# Autodesk Inventor assembly: HOATrap
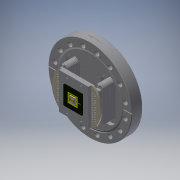
[picture p0: Inventor's stored thumbnail of the model, 180x180]
Saved by Autodesk Inventor 2016 (Build 200138000, 138)
## iProperties
Created: 2013-12-11
Part Number: HOATrap
Document SubType Name: Assembly
Designer: Michael
Author: Michael
## Documents named in this file (9)
- C:\Users\Michael\Dropbox (Personal)\Code\CAD---Experiment-systems\twins\Experiment flange\HOATrap.iam
- C:\Users\Michael\Dropbox\DO_NOT_DELETE\Flanges\Feedthroughs\Imported Components\6in_Custom_100pin\6in_Custom_100pin_Mounting_2.ipt
- C:\Users\Michael\Dropbox\DO_NOT_DELETE\UHV wiring\UHVPCB\SandiaWireRouting.ipt
- C:\Users\Michael\Dropbox\DO_NOT_DELETE\UHV wiring\mill-max-0461-3-15-15-21-XX-04-0.iam
- C:\Users\Michael\Dropbox\DO_NOT_DELETE\Flanges\Windows\Imported Components\133in_SapphireWindow_KL\133in_SapphireWindow_KL.iam
- C:\Users\Michael\Dropbox\DO_NOT_DELETE\UHV wiring\mill-max-3136-2-00-15-00-00-08-0.ipt
- C:\Users\Michael\Dropbox\DO_NOT_DELETE\Electronics\Connectors\dbConnectors\db50\db50UHV_adapter.iam
- C:\Users\Michael\Dropbox\DO_NOT_DELETE\Trap Designs\Sandia HOA Trap\HOA-Trap_Assembly.iam
- C:\Users\Michael\Dropbox (MIT)\Quanta\MG\CAD\Experiment\CavityMount.ipt
## Components (207 placed, 8 different names)
1. 6in_Custom_100pin_Mounting_2:1 — Insert:1, Angle:1, Insert:11, Insert:22, Insert:23, Insert:24, Insert:25
2. SandiaWireRouting:1 — Insert:1, Angle:1, Insert:2, Insert:12, Insert:13, Insert:14, Insert:15, Insert:16, Insert:17, Insert:18, Insert:19, Insert:20, Insert:21, Insert:28, Insert:29
3. HOA-Trap_Assembly:1 [sub-assembly] — Insert:3, Insert:4
4. 133in_SapphireWindow_KL:1 [sub-assembly] — Insert:11
5. mill-max-3136-2-00-15-00-00-08-0:50 — Insert:19
6. mill-max-3136-2-00-15-00-00-08-0:54 — Insert:18
7. mill-max-3136-2-00-15-00-00-08-0:100 — Insert:21
8. mill-max-3136-2-00-15-00-00-08-0:101 — Insert:20
9. db50UHV_adapter:1 [sub-assembly] — Insert:24, Insert:25
10. db50UHV_adapter:2 [sub-assembly] — Insert:22, Insert:23
11. CavityMount:1 — Insert:28, Insert:29
12. mill-max-0461-3-15-15-21-XX-04-0:1 [sub-assembly] — Insert:2
13. mill-max-0461-3-15-15-21-XX-04-0:2 [sub-assembly]
14. mill-max-0461-3-15-15-21-XX-04-0:3 [sub-assembly]
15. mill-max-0461-3-15-15-21-XX-04-0:4 [sub-assembly]
16. mill-max-0461-3-15-15-21-XX-04-0:5 [sub-assembly]
17. mill-max-0461-3-15-15-21-XX-04-0:6 [sub-assembly]
18. mill-max-0461-3-15-15-21-XX-04-0:7 [sub-assembly]
19. mill-max-0461-3-15-15-21-XX-04-0:8 [sub-assembly]
20. mill-max-0461-3-15-15-21-XX-04-0:9 [sub-assembly]
21. mill-max-0461-3-15-15-21-XX-04-0:10 [sub-assembly]
22. mill-max-0461-3-15-15-21-XX-04-0:11 [sub-assembly]
23. mill-max-0461-3-15-15-21-XX-04-0:12 [sub-assembly]
24. mill-max-0461-3-15-15-21-XX-04-0:13 [sub-assembly]
25. mill-max-0461-3-15-15-21-XX-04-0:14 [sub-assembly]
26. mill-max-0461-3-15-15-21-XX-04-0:15 [sub-assembly]
27. mill-max-0461-3-15-15-21-XX-04-0:16 [sub-assembly]
28. mill-max-0461-3-15-15-21-XX-04-0:17 [sub-assembly]
29. mill-max-0461-3-15-15-21-XX-04-0:18 [sub-assembly]
30. mill-max-0461-3-15-15-21-XX-04-0:19 [sub-assembly]
31. mill-max-0461-3-15-15-21-XX-04-0:20 [sub-assembly]
32. mill-max-0461-3-15-15-21-XX-04-0:21 [sub-assembly]
33. mill-max-0461-3-15-15-21-XX-04-0:22 [sub-assembly]
34. mill-max-0461-3-15-15-21-XX-04-0:23 [sub-assembly]
35. mill-max-0461-3-15-15-21-XX-04-0:24 [sub-assembly]
36. mill-max-0461-3-15-15-21-XX-04-0:25 [sub-assembly]
37. mill-max-0461-3-15-15-21-XX-04-0:26 [sub-assembly]
38. mill-max-0461-3-15-15-21-XX-04-0:27 [sub-assembly]
39. mill-max-0461-3-15-15-21-XX-04-0:28 [sub-assembly]
40. mill-max-0461-3-15-15-21-XX-04-0:32 [sub-assembly]
41. mill-max-0461-3-15-15-21-XX-04-0:33 [sub-assembly]
42. mill-max-0461-3-15-15-21-XX-04-0:34 [sub-assembly]
43. mill-max-0461-3-15-15-21-XX-04-0:38 [sub-assembly]
44. mill-max-0461-3-15-15-21-XX-04-0:39 [sub-assembly]
45. mill-max-0461-3-15-15-21-XX-04-0:40 [sub-assembly]
46. mill-max-0461-3-15-15-21-XX-04-0:41 [sub-assembly]
47. mill-max-0461-3-15-15-21-XX-04-0:51 [sub-assembly]
48. mill-max-0461-3-15-15-21-XX-04-0:52 [sub-assembly]
49. mill-max-0461-3-15-15-21-XX-04-0:53 [sub-assembly]
50. mill-max-0461-3-15-15-21-XX-04-0:54 [sub-assembly]
51. mill-max-0461-3-15-15-21-XX-04-0:64 [sub-assembly]
52. mill-max-0461-3-15-15-21-XX-04-0:65 [sub-assembly]
53. mill-max-0461-3-15-15-21-XX-04-0:66 [sub-assembly]
54. mill-max-0461-3-15-15-21-XX-04-0:67 [sub-assembly]
55. mill-max-0461-3-15-15-21-XX-04-0:68 [sub-assembly]
56. mill-max-0461-3-15-15-21-XX-04-0:76 [sub-assembly]
57. mill-max-0461-3-15-15-21-XX-04-0:77 [sub-assembly]
58. mill-max-0461-3-15-15-21-XX-04-0:78 [sub-assembly]
59. mill-max-0461-3-15-15-21-XX-04-0:79 [sub-assembly]
60. mill-max-0461-3-15-15-21-XX-04-0:80 [sub-assembly]
61. mill-max-0461-3-15-15-21-XX-04-0:81 [sub-assembly]
62. mill-max-0461-3-15-15-21-XX-04-0:89 [sub-assembly]
63. mill-max-0461-3-15-15-21-XX-04-0:90 [sub-assembly]
64. mill-max-0461-3-15-15-21-XX-04-0:91 [sub-assembly]
65. mill-max-0461-3-15-15-21-XX-04-0:92 [sub-assembly]
66. mill-max-0461-3-15-15-21-XX-04-0:93 [sub-assembly]
67. mill-max-0461-3-15-15-21-XX-04-0:94 [sub-assembly]
68. mill-max-0461-3-15-15-21-XX-04-0:102 [sub-assembly]
69. mill-max-0461-3-15-15-21-XX-04-0:103 [sub-assembly]
70. mill-max-0461-3-15-15-21-XX-04-0:104 [sub-assembly]
71. mill-max-0461-3-15-15-21-XX-04-0:105 [sub-assembly]
72. mill-max-0461-3-15-15-21-XX-04-0:106 [sub-assembly]
73. mill-max-0461-3-15-15-21-XX-04-0:116 [sub-assembly]
74. mill-max-0461-3-15-15-21-XX-04-0:117 [sub-assembly]
75. mill-max-0461-3-15-15-21-XX-04-0:118 [sub-assembly]
76. mill-max-0461-3-15-15-21-XX-04-0:119 [sub-assembly]
77. mill-max-0461-3-15-15-21-XX-04-0:129 [sub-assembly]
78. mill-max-0461-3-15-15-21-XX-04-0:130 [sub-assembly]
79. mill-max-0461-3-15-15-21-XX-04-0:131 [sub-assembly]
80. mill-max-0461-3-15-15-21-XX-04-0:132 [sub-assembly]
81. mill-max-0461-3-15-15-21-XX-04-0:136 [sub-assembly]
82. mill-max-0461-3-15-15-21-XX-04-0:137 [sub-assembly]
83. mill-max-0461-3-15-15-21-XX-04-0:138 [sub-assembly]
84. mill-max-0461-3-15-15-21-XX-04-0:142 [sub-assembly]
85. mill-max-0461-3-15-15-21-XX-04-0:143 [sub-assembly]
86. mill-max-0461-3-15-15-21-XX-04-0:144 [sub-assembly]
87. mill-max-0461-3-15-15-21-XX-04-0:145 [sub-assembly]
88. mill-max-0461-3-15-15-21-XX-04-0:146 [sub-assembly]
89. mill-max-0461-3-15-15-21-XX-04-0:147 [sub-assembly]
90. mill-max-0461-3-15-15-21-XX-04-0:148 [sub-assembly]
91. mill-max-0461-3-15-15-21-XX-04-0:149 [sub-assembly]
92. mill-max-0461-3-15-15-21-XX-04-0:150 [sub-assembly]
93. mill-max-0461-3-15-15-21-XX-04-0:151 [sub-assembly]
94. mill-max-0461-3-15-15-21-XX-04-0:152 [sub-assembly]
95. mill-max-0461-3-15-15-21-XX-04-0:153 [sub-assembly]
96. mill-max-0461-3-15-15-21-XX-04-0:154 [sub-assembly]
97. mill-max-0461-3-15-15-21-XX-04-0:155 [sub-assembly]
98. mill-max-0461-3-15-15-21-XX-04-0:156 [sub-assembly]
99. mill-max-0461-3-15-15-21-XX-04-0:157 [sub-assembly] — Insert:3
100. mill-max-0461-3-15-15-21-XX-04-0:158 [sub-assembly]
101. mill-max-0461-3-15-15-21-XX-04-0:159 [sub-assembly]
102. mill-max-0461-3-15-15-21-XX-04-0:160 [sub-assembly]
103. mill-max-0461-3-15-15-21-XX-04-0:161 [sub-assembly]
104. mill-max-0461-3-15-15-21-XX-04-0:162 [sub-assembly]
105. mill-max-0461-3-15-15-21-XX-04-0:163 [sub-assembly]
106. mill-max-0461-3-15-15-21-XX-04-0:164 [sub-assembly]
107. mill-max-0461-3-15-15-21-XX-04-0:165 [sub-assembly]
108. mill-max-0461-3-15-15-21-XX-04-0:166 [sub-assembly]
109. mill-max-0461-3-15-15-21-XX-04-0:167 [sub-assembly]
110. mill-max-0461-3-15-15-21-XX-04-0:168 [sub-assembly]
111. mill-max-0461-3-15-15-21-XX-04-0:169 [sub-assembly] — Insert:4
112. mill-max-3136-2-00-15-00-00-08-0:4 — Insert:14
113. mill-max-3136-2-00-15-00-00-08-0:3 — Insert:13
114. mill-max-3136-2-00-15-00-00-08-0:2 — Insert:12
115. mill-max-3136-2-00-15-00-00-08-0:5
116. mill-max-3136-2-00-15-00-00-08-0:6
117. mill-max-3136-2-00-15-00-00-08-0:7
118. mill-max-3136-2-00-15-00-00-08-0:8
119. mill-max-3136-2-00-15-00-00-08-0:9
120. mill-max-3136-2-00-15-00-00-08-0:10
121. mill-max-3136-2-00-15-00-00-08-0:11
122. mill-max-3136-2-00-15-00-00-08-0:12
123. mill-max-3136-2-00-15-00-00-08-0:13
124. mill-max-3136-2-00-15-00-00-08-0:14
125. mill-max-3136-2-00-15-00-00-08-0:15
126. mill-max-3136-2-00-15-00-00-08-0:16
127. mill-max-3136-2-00-15-00-00-08-0:17
128. mill-max-3136-2-00-15-00-00-08-0:18
129. mill-max-3136-2-00-15-00-00-08-0:19
130. mill-max-3136-2-00-15-00-00-08-0:20
131. mill-max-3136-2-00-15-00-00-08-0:21
132. mill-max-3136-2-00-15-00-00-08-0:22
133. mill-max-3136-2-00-15-00-00-08-0:23
134. mill-max-3136-2-00-15-00-00-08-0:24
135. mill-max-3136-2-00-15-00-00-08-0:25
136. mill-max-3136-2-00-15-00-00-08-0:26
137. mill-max-3136-2-00-15-00-00-08-0:27
138. mill-max-3136-2-00-15-00-00-08-0:28
139. mill-max-3136-2-00-15-00-00-08-0:29
140. mill-max-3136-2-00-15-00-00-08-0:30
141. mill-max-3136-2-00-15-00-00-08-0:31
142. mill-max-3136-2-00-15-00-00-08-0:32
143. mill-max-3136-2-00-15-00-00-08-0:33
144. mill-max-3136-2-00-15-00-00-08-0:34
145. mill-max-3136-2-00-15-00-00-08-0:35
146. mill-max-3136-2-00-15-00-00-08-0:36
147. mill-max-3136-2-00-15-00-00-08-0:37
148. mill-max-3136-2-00-15-00-00-08-0:38
149. mill-max-3136-2-00-15-00-00-08-0:39
150. mill-max-3136-2-00-15-00-00-08-0:40
151. mill-max-3136-2-00-15-00-00-08-0:41
152. mill-max-3136-2-00-15-00-00-08-0:42
153. mill-max-3136-2-00-15-00-00-08-0:43
154. mill-max-3136-2-00-15-00-00-08-0:44
155. mill-max-3136-2-00-15-00-00-08-0:45
156. mill-max-3136-2-00-15-00-00-08-0:46
157. mill-max-3136-2-00-15-00-00-08-0:47
158. mill-max-3136-2-00-15-00-00-08-0:48
159. mill-max-3136-2-00-15-00-00-08-0:49
160. mill-max-3136-2-00-15-00-00-08-0:52 — Insert:15
161. mill-max-3136-2-00-15-00-00-08-0:53 — Insert:16
162. mill-max-3136-2-00-15-00-00-08-0:51 — Insert:17
163. mill-max-3136-2-00-15-00-00-08-0:55
164. mill-max-3136-2-00-15-00-00-08-0:56
165. mill-max-3136-2-00-15-00-00-08-0:57
166. mill-max-3136-2-00-15-00-00-08-0:58
167. mill-max-3136-2-00-15-00-00-08-0:59
168. mill-max-3136-2-00-15-00-00-08-0:60
169. mill-max-3136-2-00-15-00-00-08-0:61
170. mill-max-3136-2-00-15-00-00-08-0:62
171. mill-max-3136-2-00-15-00-00-08-0:63
172. mill-max-3136-2-00-15-00-00-08-0:64
173. mill-max-3136-2-00-15-00-00-08-0:65
174. mill-max-3136-2-00-15-00-00-08-0:66
175. mill-max-3136-2-00-15-00-00-08-0:67
176. mill-max-3136-2-00-15-00-00-08-0:68
177. mill-max-3136-2-00-15-00-00-08-0:69
178. mill-max-3136-2-00-15-00-00-08-0:70
179. mill-max-3136-2-00-15-00-00-08-0:71
180. mill-max-3136-2-00-15-00-00-08-0:72
181. mill-max-3136-2-00-15-00-00-08-0:73
182. mill-max-3136-2-00-15-00-00-08-0:74
183. mill-max-3136-2-00-15-00-00-08-0:75
184. mill-max-3136-2-00-15-00-00-08-0:76
185. mill-max-3136-2-00-15-00-00-08-0:77
186. mill-max-3136-2-00-15-00-00-08-0:78
187. mill-max-3136-2-00-15-00-00-08-0:79
188. mill-max-3136-2-00-15-00-00-08-0:80
189. mill-max-3136-2-00-15-00-00-08-0:81
190. mill-max-3136-2-00-15-00-00-08-0:82
191. mill-max-3136-2-00-15-00-00-08-0:83
192. mill-max-3136-2-00-15-00-00-08-0:84
193. mill-max-3136-2-00-15-00-00-08-0:85
194. mill-max-3136-2-00-15-00-00-08-0:86
195. mill-max-3136-2-00-15-00-00-08-0:87
196. mill-max-3136-2-00-15-00-00-08-0:88
197. mill-max-3136-2-00-15-00-00-08-0:89
198. mill-max-3136-2-00-15-00-00-08-0:90
199. mill-max-3136-2-00-15-00-00-08-0:91
200. mill-max-3136-2-00-15-00-00-08-0:92
201. mill-max-3136-2-00-15-00-00-08-0:93
202. mill-max-3136-2-00-15-00-00-08-0:94
203. mill-max-3136-2-00-15-00-00-08-0:95
204. mill-max-3136-2-00-15-00-00-08-0:96
205. mill-max-3136-2-00-15-00-00-08-0:97
206. mill-max-3136-2-00-15-00-00-08-0:98
207. mill-max-3136-2-00-15-00-00-08-0:99
## Component patterns: (169 elements, first: mill-max-0461-3-15-15-21-XX-04-0:1), (16 elements, first: mill-max-3136-2-00-15-00-00-08-0:4 + mill-max-3136-2-00-15-00-00-08-0:3 + mill-max-3136-2-00-15-00-00-08-0:2), (16 elements, first: mill-max-3136-2-00-15-00-00-08-0:52 + mill-max-3136-2-00-15-00-00-08-0:53 + mill-max-3136-2-00-15-00-00-08-0:51)
## Relationships (22: Insert 21, Angle 1)
- Insert:1 (22.86 mm): 6in_Custom_100pin_Mounting_2:1 ↔ SandiaWireRouting:1
- Angle:1 (90 deg): 6in_Custom_100pin_Mounting_2:1 ↔ SandiaWireRouting:1
- Insert:2: SandiaWireRouting:1 ↔ mill-max-0461-3-15-15-21-XX-04-0:1
- Insert:3: HOA-Trap_Assembly:1 ↔ mill-max-0461-3-15-15-21-XX-04-0:157
- Insert:4: HOA-Trap_Assembly:1 ↔ mill-max-0461-3-15-15-21-XX-04-0:169
- Insert:11: 6in_Custom_100pin_Mounting_2:1 ↔ 133in_SapphireWindow_KL:1
- Insert:12: SandiaWireRouting:1 ↔ mill-max-3136-2-00-15-00-00-08-0:2
- Insert:13: SandiaWireRouting:1 ↔ mill-max-3136-2-00-15-00-00-08-0:3
- Insert:14: SandiaWireRouting:1 ↔ mill-max-3136-2-00-15-00-00-08-0:4
- Insert:15: SandiaWireRouting:1 ↔ mill-max-3136-2-00-15-00-00-08-0:52
- Insert:16: SandiaWireRouting:1 ↔ mill-max-3136-2-00-15-00-00-08-0:53
- Insert:17: SandiaWireRouting:1 ↔ mill-max-3136-2-00-15-00-00-08-0:51
- Insert:18: SandiaWireRouting:1 ↔ mill-max-3136-2-00-15-00-00-08-0:54
- Insert:19: SandiaWireRouting:1 ↔ mill-max-3136-2-00-15-00-00-08-0:50
- Insert:20: SandiaWireRouting:1 ↔ mill-max-3136-2-00-15-00-00-08-0:101
- Insert:21: SandiaWireRouting:1 ↔ mill-max-3136-2-00-15-00-00-08-0:100
- Insert:22: 6in_Custom_100pin_Mounting_2:1 ↔ db50UHV_adapter:2
- Insert:23: 6in_Custom_100pin_Mounting_2:1 ↔ db50UHV_adapter:2
- Insert:24: 6in_Custom_100pin_Mounting_2:1 ↔ db50UHV_adapter:1
- Insert:25: 6in_Custom_100pin_Mounting_2:1 ↔ db50UHV_adapter:1
- Insert:28: SandiaWireRouting:1 ↔ CavityMount:1
- Insert:29: SandiaWireRouting:1 ↔ CavityMount:1
